# Autodesk Inventor assembly: GimbalMotor
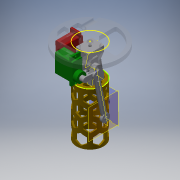
[picture p0: Inventor's stored thumbnail of the model, 180x180]
Saved by Autodesk Inventor 2018 (Build 220112000, 112)
## iProperties
Created: 2020-03-22
Part Number: GimbalMotor
Document SubType Name: Assembly
Designer: technik
Author: technik
## Documents named in this file (8)
- E:\repos-f\astro\ranger\cad\GimbalMotor.iam
- E:\repos-f\astro\ranger\cad\servoPlate.ipt
- E:\repos-f\astro\ranger\cad\DoubleCardan.iam
- E:\repos-f\astro\ranger\cad\MotorCase.ipt
- E:\repos-f\astro\ranger\cad\MicroServo.ipt
- E:\repos-f\astro\ranger\cad\ServoArm.ipt
- E:\repos-f\astro\ranger\cad\BackArm.ipt
- E:\repos-f\astro\ranger\cad\ballJoint.ipt
## Components (11 placed, 7 different names)
1. servoPlate:1 — Flush:1, Flush:2, Flush:3, Mate:1, Mate:2, Mate:19, Mate:20
2. DoubleCardan:1 [sub-assembly] — Mate:1, Mate:2, Mate:3, Angle:1, Mate:4, Angle:2
3. MotorCase:1 — Mate:3, Mate:4, Angle:2, Angle:3, Tangent:1, Angle:4, Tangent:2, Mate:15, Mate:16
4. MicroServo:1 — Mate:7, Mate:8, Mate:20
5. MicroServo:2 — Mate:9, Mate:10, Mate:19
6. ServoArm:1 — Mate:7, Mate:8, Flush:5, Mate:17
7. ServoArm:2 — Mate:9, Mate:10, Flush:4, Mate:11, Mate:12
8. BackArm:1 — Mate:11, Mate:12
9. ballJoint:1 — Mate:14, Mate:15
10. ballJoint:2 — Mate:13, Mate:16, Mate:18
11. BackArm:2 — Mate:17, Mate:18
## Relationships (29: Mate 18, Flush 5, Angle 4, Tangent 2)
- Flush:1: servoPlate:1
- Flush:2: servoPlate:1
- Flush:3: servoPlate:1
- Mate:1: servoPlate:1 ↔ DoubleCardan:1
- Mate:2: servoPlate:1 ↔ DoubleCardan:1
- Mate:3: DoubleCardan:1 ↔ MotorCase:1
- Angle:1 (0 deg): DoubleCardan:1
- Mate:4: DoubleCardan:1 ↔ MotorCase:1
- Angle:2 (0 deg): DoubleCardan:1 ↔ MotorCase:1
- Angle:3 (0 deg): MotorCase:1
- Tangent:1: MotorCase:1
- Angle:4 (0 deg): MotorCase:1
- Tangent:2: MotorCase:1
- Mate:7: MicroServo:1 ↔ ServoArm:1
- Mate:8: MicroServo:1 ↔ ServoArm:1
- Mate:9: MicroServo:2 ↔ ServoArm:2
- Mate:10: MicroServo:2 ↔ ServoArm:2
- Flush:4: ServoArm:2
- Flush:5: ServoArm:1
- Mate:11: ServoArm:2 ↔ BackArm:1
- Mate:12: ServoArm:2 ↔ BackArm:1
- Mate:13: ballJoint:2
- Mate:14: ballJoint:1
- Mate:15: MotorCase:1 ↔ ballJoint:1
- Mate:16: MotorCase:1 ↔ ballJoint:2
- Mate:17: ServoArm:1 ↔ BackArm:2
- Mate:18: ballJoint:2 ↔ BackArm:2
- Mate:19: servoPlate:1 ↔ MicroServo:2
- Mate:20: servoPlate:1 ↔ MicroServo:1
